# Autodesk Inventor assembly: RotatingBase
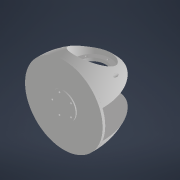
[picture p0: Inventor's stored thumbnail of the model, 180x180]
Saved by Autodesk Inventor 2021 (Build 250183000, 183)
## iProperties
Created: 2022-10-01
Part Number: RotatingBase
Document SubType Name: Assembly
Designer: MicnedSQ
Author: MicnedSQ
## Documents named in this file (4)
- C:\Users\MicnedSQ\Desktop\V1\RotatingBase\RotatingBase.iam
- C:\Users\MicnedSQ\Desktop\V1\RotatingBase\Bottom.ipt
- C:\Users\MicnedSQ\Desktop\V1\RotatingBase\Left.ipt
- C:\Users\MicnedSQ\Desktop\V1\RotatingBase\Right.ipt
## Components (3 placed, 3 different names)
1. Bottom:1 — Sztywne:1, Sztywne:2
2. Left:1 — Sztywne:1
3. Right:1 — Sztywne:2
## Relationships (2: WeldJoint 2)
- Sztywne:1 [WeldJoint]: Bottom:1 ↔ Left:1
- Sztywne:2 [WeldJoint]: Bottom:1 ↔ Right:1
